# Autodesk Inventor assembly: ASY MSC 203 RIGHT BOARD
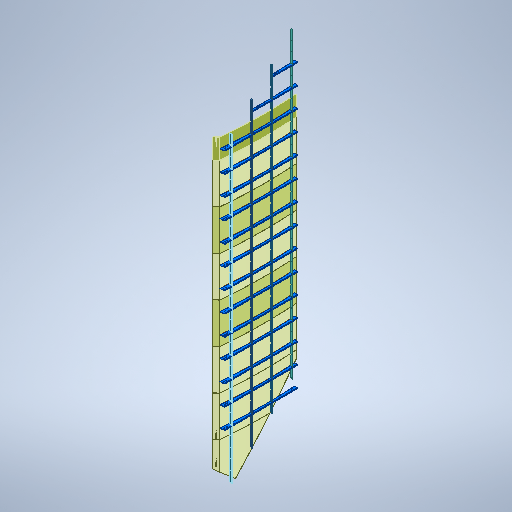
[picture p0: Inventor's stored thumbnail of the model, 512x512]
Saved by Autodesk Inventor 2025 (Build 290162010, 162A)
## iProperties
Created: 2024-07-22
Part Number: ASY MSC 203 RIGHT BOARD
Document SubType Name: Assembly
Designer: pokla
Author: pokla
## Documents named in this file (13)
- C:\Users\pokla\Documents\Inventor\Отстойник осветлитель\Manturovo_Se-clar-Gleb\ASY MSC 203 RIGHT BOARD.iam
- C:\Users\pokla\Documents\Inventor\Отстойник осветлитель\Manturovo_Se-clar-Gleb\MSC 052 rib board.ipt
- C:\Users\pokla\Documents\Inventor\Отстойник осветлитель\Manturovo_Se-clar-Gleb\MSC 024 sheet board main.ipt
- C:\Users\pokla\Documents\Inventor\Отстойник осветлитель\Manturovo_Se-clar-Gleb\MSC 023 sheet board.ipt
- C:\Users\pokla\Documents\Inventor\Отстойник осветлитель\Manturovo_Se-clar-Gleb\MSC 063 stringer board #.ipt
- C:\Users\pokla\Documents\Inventor\Отстойник осветлитель\Manturovo_Se-clar-Gleb\MSC 064 stringer board ##.ipt
- C:\Users\pokla\Documents\Inventor\Отстойник осветлитель\Manturovo_Se-clar-Gleb\MSC 065 stringer board ###.ipt
- C:\Users\pokla\Documents\Inventor\Отстойник осветлитель\Manturovo_Se-clar-Gleb\MSC 066 stringer board ####.ipt
- C:\Users\pokla\Documents\Inventor\Отстойник осветлитель\Manturovo_Se-clar-Gleb\MSC 026 sheet board withers 2.ipt
- C:\Users\pokla\Documents\Inventor\Отстойник осветлитель\Manturovo_Se-clar-Gleb\MSC 028 sheet board face 2.ipt
- C:\Users\pokla\Documents\Inventor\Отстойник осветлитель\Manturovo_Se-clar-Gleb\MSC 055 rib hip 2.ipt
- C:\Users\pokla\Documents\Inventor\Отстойник осветлитель\Manturovo_Se-clar-Gleb\MSC 054 rib hip 1.ipt
- C:\Users\pokla\Documents\Inventor\Отстойник осветлитель\Manturovo_Se-clar-Gleb\MSC 0512 rib back mould .ipt
## Components (55 placed, 17 different names)
1. MSC 052 rib board.ipt:1 — Rigid:16, Rigid:17
2. MSC 024 sheet board main.ipt:6
3. MSC 024 sheet board main.ipt:7
4. MSC 024 sheet board main.ipt:8
5. MSC 024 sheet board main.ipt:9
6. MSC 024 sheet board main.ipt:10 — Flush:2, Flush:3, Flush:4
7. MSC 023 sheet board.ipt:2
8. MSC 063 stringer board #.ipt:1
9. MSC 064 stringer board ##.ipt:1
10. MSC 065 stringer board ###.ipt:1
11. MSC 066 stringer board ####.ipt:1
12. MSC 026 sheet board withers 2.ipt:1
13. MSC 028 sheet board face 2.ipt:1
14. MSC 052 rib board.ipt:4 — Rigid:16, Flush:1, Flush:2, Flush:3, Rigid:31
15. MSC 063 stringer board #.ipt:4 — Rigid:19
16. MSC 064 stringer board ##.ipt:4 — Rigid:22
17. MSC 065 stringer board ###.ipt:4 — Rigid:25
18. MSC 066 stringer board ####.ipt:4 — Rigid:28
19. MSC 055 rib hip 2:1 — Rigid:17, Rigid:18
20. MSC 054 rib board hip 1:1 — Rigid:18
21. MSC 0512 rib back mould :1 — Flush:4, Flush:5, Flush:6, Rigid:42, Rigid:43
22. МОО 053 стрингер борт 3:3 — Rigid:19, Rigid:20
23. МОО 053 стрингер борт 3:5 — Rigid:20, Rigid:21
24. МОО 053 стрингер борт 3:6 — Rigid:21
25. МОО 054 стрингер борт 4:3 — Rigid:22, Rigid:23
26. МОО 054 стрингер борт 4:5 — Rigid:23, Rigid:24
27. МОО 054 стрингер борт 4:6 — Rigid:24
28. МОО 055 стрингер борт 5:3 — Rigid:25, Rigid:26
29. МОО 055 стрингер борт 5:5 — Rigid:26, Rigid:27
30. МОО 055 стрингер борт 5:6 — Rigid:27
31. МОО 056 стрингер борт 6:3 — Rigid:28, Rigid:29
32. МОО 056 стрингер борт 6:5 — Rigid:29, Rigid:30
33. МОО 056 стрингер борт 6:6 — Rigid:30
34. MSC 052 rib board:3 — Rigid:31, Rigid:32
35. MSC 052 rib board:5 — Rigid:32, Rigid:33
36. MSC 052 rib board:6 — Rigid:33, Rigid:34
37. MSC 052 rib board:7 — Rigid:34, Rigid:38
38. MSC 052 rib board:8 — Rigid:38
39. MSC 052 rib board:9
40. MSC 052 rib board:10
41. MSC 052 rib board:11 — Rigid:41
42. MSC 052 rib board:12 — Rigid:41
43. MSC 052 rib board:13
44. MSC 052 rib board:14
45. MSC 0512 rib back mould :2 — Rigid:42
46. MSC 0512 rib back mould :3 — Rigid:43, Rigid:44
47. MSC 0512 rib back mould :4 — Rigid:44, Rigid:45
48. MSC 0512 rib back mould :5 — Rigid:45, Rigid:48
49. MSC 0512 rib back mould :6 — Rigid:48
50. MSC 0512 rib back mould :7
51. MSC 0512 rib back mould :8 — Rigid:54
52. MSC 0512 rib back mould :9 — Rigid:54
53. MSC 0512 rib back mould :10
54. MSC 0512 rib back mould :11
55. MSC 0512 rib back mould :12
## Relationships (58: WeldJoint 52, Flush 6)
- [WeldJoint]: MSC 024 sheet board main.ipt:6 ↔ MSC 024 sheet board main.ipt:7
- [WeldJoint]: MSC 024 sheet board main.ipt:7 ↔ MSC 024 sheet board main.ipt:8
- [WeldJoint]: MSC 024 sheet board main.ipt:8 ↔ MSC 024 sheet board main.ipt:9
- [WeldJoint]: MSC 024 sheet board main.ipt:9 ↔ MSC 024 sheet board main.ipt:10
- [WeldJoint]: MSC 024 sheet board main.ipt:10 ↔ MSC 023 sheet board.ipt:2
- [WeldJoint]: MSC 026 sheet board withers 2.ipt:1 ↔ MSC 028 sheet board face 2.ipt:1
- [WeldJoint]: MSC 024 sheet board main.ipt:6 ↔ MSC 026 sheet board withers 2.ipt:1
- [WeldJoint]: MSC 063 stringer board #.ipt:1 ↔ MSC 063 stringer board #.ipt:4
- [WeldJoint]: MSC 064 stringer board ##.ipt:1 ↔ MSC 064 stringer board ##.ipt:4
- [WeldJoint]: MSC 065 stringer board ###.ipt:1 ↔ MSC 065 stringer board ###.ipt:4
- [WeldJoint]: MSC 066 stringer board ####.ipt:1 ↔ MSC 066 stringer board ####.ipt:4
- [WeldJoint] (2 mm): MSC 052 rib board.ipt:1 ↔ MSC 063 stringer board #.ipt:4
- [WeldJoint] (2 mm): MSC 052 rib board.ipt:1 ↔ MSC 066 stringer board ####.ipt:1
- [WeldJoint] (2 mm): MSC 052 rib board.ipt:1 ↔ MSC 065 stringer board ###.ipt:1
- [WeldJoint] (2 mm): MSC 052 rib board.ipt:1 ↔ MSC 064 stringer board ##.ipt:1
- Rigid:16 [WeldJoint] (-500 mm): MSC 052 rib board.ipt:1 ↔ MSC 052 rib board.ipt:4
- Rigid:17 [WeldJoint] (500 mm): MSC 052 rib board.ipt:1 ↔ MSC 055 rib hip 2:1
- Rigid:18 [WeldJoint] (500 mm): MSC 055 rib hip 2:1 ↔ MSC 054 rib board hip 1:1
- Flush:1: MSC 052 rib board.ipt:4
- Flush:2 (250 mm): MSC 024 sheet board main.ipt:10 ↔ MSC 052 rib board.ipt:4
- Flush:3: MSC 024 sheet board main.ipt:10 ↔ MSC 052 rib board.ipt:4
- Rigid:19 [WeldJoint]: MSC 063 stringer board #.ipt:4 ↔ МОО 053 стрингер борт 3:3
- Rigid:20 [WeldJoint]: МОО 053 стрингер борт 3:3 ↔ МОО 053 стрингер борт 3:5
- Rigid:21 [WeldJoint]: МОО 053 стрингер борт 3:5 ↔ МОО 053 стрингер борт 3:6
- Rigid:22 [WeldJoint]: MSC 064 stringer board ##.ipt:4 ↔ МОО 054 стрингер борт 4:3
- Rigid:23 [WeldJoint]: МОО 054 стрингер борт 4:3 ↔ МОО 054 стрингер борт 4:5
- Rigid:24 [WeldJoint]: МОО 054 стрингер борт 4:5 ↔ МОО 054 стрингер борт 4:6
- Rigid:25 [WeldJoint]: MSC 065 stringer board ###.ipt:4 ↔ МОО 055 стрингер борт 5:3
- Rigid:26 [WeldJoint]: МОО 055 стрингер борт 5:3 ↔ МОО 055 стрингер борт 5:5
- Rigid:27 [WeldJoint]: МОО 055 стрингер борт 5:5 ↔ МОО 055 стрингер борт 5:6
- Rigid:28 [WeldJoint]: MSC 066 stringer board ####.ipt:4 ↔ МОО 056 стрингер борт 6:3
- Rigid:29 [WeldJoint]: МОО 056 стрингер борт 6:3 ↔ МОО 056 стрингер борт 6:5
- Rigid:30 [WeldJoint]: МОО 056 стрингер борт 6:5 ↔ МОО 056 стрингер борт 6:6
- Rigid:31 [WeldJoint] (-500 mm): MSC 052 rib board.ipt:4 ↔ MSC 052 rib board:3
- Rigid:32 [WeldJoint] (-500 mm): MSC 052 rib board:3 ↔ MSC 052 rib board:5
- Rigid:33 [WeldJoint] (-500 mm): MSC 052 rib board:5 ↔ MSC 052 rib board:6
- Rigid:34 [WeldJoint] (-500 mm): MSC 052 rib board:6 ↔ MSC 052 rib board:7
- [WeldJoint] (-500 mm): MSC 052 rib board:8 ↔ MSC 052 rib board:9
- [WeldJoint] (-500 mm): MSC 052 rib board:9 ↔ MSC 052 rib board:10
- [WeldJoint] (-500 mm): MSC 052 rib board:10 ↔ MSC 052 rib board:11
- Rigid:38 [WeldJoint] (-500 mm): MSC 052 rib board:7 ↔ MSC 052 rib board:8
- [WeldJoint] (-500 mm): MSC 052 rib board:12 ↔ MSC 052 rib board:13
- [WeldJoint] (-500 mm): MSC 052 rib board:13 ↔ MSC 052 rib board:14
- Rigid:41 [WeldJoint] (-500 mm): MSC 052 rib board:11 ↔ MSC 052 rib board:12
- Flush:4 (248.5 mm): MSC 024 sheet board main.ipt:10 ↔ MSC 0512 rib back mould :1
- Flush:5: MSC 0512 rib back mould :1
- Flush:6: MSC 0512 rib back mould :1
- Rigid:42 [WeldJoint] (497 mm): MSC 0512 rib back mould :1 ↔ MSC 0512 rib back mould :2
- Rigid:43 [WeldJoint] (497 mm): MSC 0512 rib back mould :1 ↔ MSC 0512 rib back mould :3
- Rigid:44 [WeldJoint] (497 mm): MSC 0512 rib back mould :3 ↔ MSC 0512 rib back mould :4
- Rigid:45 [WeldJoint] (497 mm): MSC 0512 rib back mould :4 ↔ MSC 0512 rib back mould :5
- [WeldJoint] (497 mm): MSC 0512 rib back mould :6 ↔ MSC 0512 rib back mould :7
- [WeldJoint] (497 mm): MSC 0512 rib back mould :7 ↔ MSC 0512 rib back mould :8
- Rigid:48 [WeldJoint] (497 mm): MSC 0512 rib back mould :5 ↔ MSC 0512 rib back mould :6
- [WeldJoint] (497 mm): MSC 0512 rib back mould :9 ↔ MSC 0512 rib back mould :10
- [WeldJoint] (497 mm): MSC 0512 rib back mould :10 ↔ MSC 0512 rib back mould :11
- [WeldJoint] (497 mm): MSC 0512 rib back mould :11 ↔ MSC 0512 rib back mould :12
- Rigid:54 [WeldJoint] (497 mm): MSC 0512 rib back mould :8 ↔ MSC 0512 rib back mould :9
## Named parameters: d230_d194 = 0 mm, d231_d195 = 0 mm, d232_d160 = 0 mm, d233_d161 = 0 mm, d39_d36 = -500 mm, d40_d37 = -500 mm, d41_d38 = -500 mm, d43_d40_d37 = -500 mm, d44_d41_d38 = -500 mm, d53_d51 = 497 mm, d54_d52 = 497 mm, d56_d51 = 497 mm, d57_d52 = 497 mm, d60_d55 = 497 mm
